# Autodesk Inventor assembly: 000.010 - Крышка
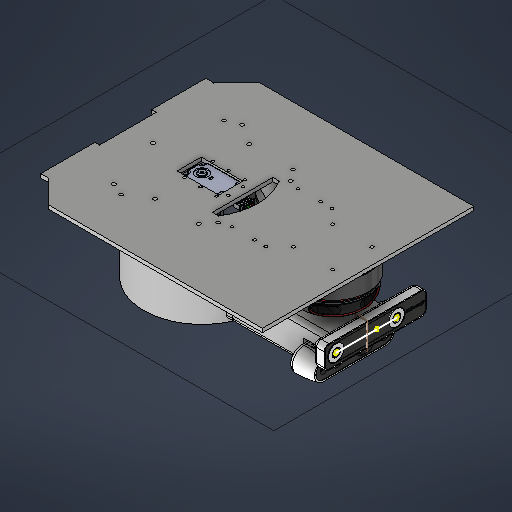
[picture p0: Inventor's stored thumbnail of the model, 512x512]
Saved by Autodesk Inventor 2025 (Build 290162000, 162)
## iProperties
Created: 2024-08-22
Part Number: 000.010 - Крышка
Document SubType Name: Assembly
Designer: IvanPetrov
Author: IvanPetrov
## Documents named in this file (10)
- D:\Projects\OmniBot\design\000.010 - Крышка.iam
- D:\Projects\OmniBot\design\000.010.001 - Секция центральная.ipt
- D:\Projects\OmniBot\design\000.010.002 - Основание манипулятора.ipt
- D:\Projects\OmniBot\design\Манипулятор AR\28Tyy.ipt
- D:\Projects\OmniBot\design\000.010.003 - Кожух.ipt
- D:\Projects\OmniBot\design\000.010.003 - Кожухзеркальный.ipt
- D:\Projects\OmniBot\design\standart_components\Realsense\D400\IntelRealsense_D435_Multibody.ipt
- D:\Projects\OmniBot\design\standart_components\Realsense\D200\Intel RealSense T265.iam
- D:\Projects\OmniBot\design\standart_components\Lidar\RPLIDAR A2.iam
- D:\Projects\OmniBot\design\000.010.004 - Крепление камер.ipt
## Components (9 placed, 9 different names)
1. 000.010.001 - Секция центральная:1 — Совмещение:1, Угол:1, Заподлицо:1, Совмещение:3, Совмещение:6, Совмещение:13, Угол:3, Касательность:1, Совмещение:15
2. 000.010.002 - Основание манипулятора:1 — Совмещение:1, Угол:1, Заподлицо:1, Совмещение:2, Совмещение:4, Совмещение:5, Заподлицо:2, Совмещение:8
3. 28Tyy:1 — Совмещение:3, Совмещение:4, Совмещение:5, Заподлицо:2, Совмещение:7
4. 000.010.003 - Кожух:1 — Совмещение:6, Совмещение:7, Совмещение:8, Касательность:2
5. 000.010.003 - Кожухзеркальный:1
6. IntelRealsense_D435_Multibody:1 — Угол:2, Совмещение:11, Совмещение:12, Совмещение:17, Совмещение:18, Совмещение:19
7. Intel RealSense T265:1 [sub-assembly] — Угол:2, Совмещение:11, Заподлицо:3, Совмещение:12, Совмещение:14
8. RPLIDAR A2:1 [sub-assembly] — Совмещение:13, Угол:3, Совмещение:14, Касательность:1
9. 000.010.004 - Крепление камер:1 — Совмещение:15, Касательность:2, Совмещение:16, Совмещение:17, Совмещение:18, Совмещение:19
## Relationships (25: Mate 17, Angle 3, Flush 3, Tangent 2)
- Совмещение:1 [Mate]: 000.010.001 - Секция центральная:1 ↔ 000.010.002 - Основание манипулятора:1
- Угол:1 [Angle] (0 deg): 000.010.001 - Секция центральная:1 ↔ 000.010.002 - Основание манипулятора:1
- Заподлицо:1 [Flush] (40.5 mm): 000.010.001 - Секция центральная:1 ↔ 000.010.002 - Основание манипулятора:1
- Совмещение:2 [Mate]: 000.010.002 - Основание манипулятора:1
- Совмещение:3 [Mate]: 000.010.001 - Секция центральная:1 ↔ 28Tyy:1
- Совмещение:4 [Mate]: 000.010.002 - Основание манипулятора:1 ↔ 28Tyy:1
- Совмещение:5 [Mate]: 000.010.002 - Основание манипулятора:1 ↔ 28Tyy:1
- Заподлицо:2 [Flush] (4.4 mm): 000.010.002 - Основание манипулятора:1 ↔ 28Tyy:1
- Совмещение:6 [Mate]: 000.010.001 - Секция центральная:1 ↔ 000.010.003 - Кожух:1
- Совмещение:7 [Mate]: 28Tyy:1 ↔ 000.010.003 - Кожух:1
- Совмещение:8 [Mate]: 000.010.002 - Основание манипулятора:1 ↔ 000.010.003 - Кожух:1
- Угол:2 [Angle] (0 deg): IntelRealsense_D435_Multibody:1 ↔ Intel RealSense T265:1
- Совмещение:11 [Mate]: IntelRealsense_D435_Multibody:1 ↔ Intel RealSense T265:1
- Заподлицо:3 [Flush]: Intel RealSense T265:1
- Совмещение:12 [Mate]: IntelRealsense_D435_Multibody:1 ↔ Intel RealSense T265:1
- Совмещение:13 [Mate]: 000.010.001 - Секция центральная:1 ↔ RPLIDAR A2:1
- Угол:3 [Angle] (180 deg): 000.010.001 - Секция центральная:1 ↔ RPLIDAR A2:1
- Совмещение:14 [Mate]: Intel RealSense T265:1 ↔ RPLIDAR A2:1
- Касательность:1 [Tangent]: 000.010.001 - Секция центральная:1 ↔ RPLIDAR A2:1
- Совмещение:15 [Mate]: 000.010.001 - Секция центральная:1 ↔ 000.010.004 - Крепление камер:1
- Касательность:2 [Tangent]: 000.010.003 - Кожух:1 ↔ 000.010.004 - Крепление камер:1
- Совмещение:16 [Mate]: 000.010.004 - Крепление камер:1
- Совмещение:17 [Mate]: IntelRealsense_D435_Multibody:1 ↔ 000.010.004 - Крепление камер:1
- Совмещение:18 [Mate]: IntelRealsense_D435_Multibody:1 ↔ 000.010.004 - Крепление камер:1
- Совмещение:19 [Mate] (3 mm): IntelRealsense_D435_Multibody:1 ↔ 000.010.004 - Крепление камер:1
